# Autodesk Inventor assembly: Full Project Assembly
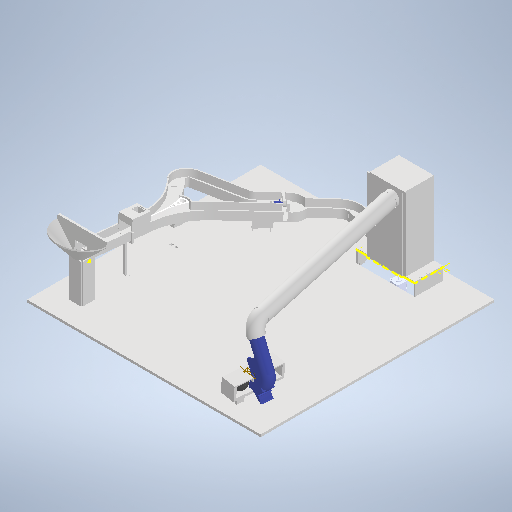
[picture p0: Inventor's stored thumbnail of the model, 512x512]
Saved by Autodesk Inventor 2025.3 (Build 293356000, 356)
## iProperties
Created: 2026-04-18
Part Number: Full Project Assembly
Document SubType Name: Assembly
Designer: kamal
Author: kamal
## Documents named in this file (21)
- C:\Users\kamal\OneDrive\Desktop\Personal\semester 4\Basics of Mechatronics\Full Assembly\Full Project Assembly.iam
- C:\Users\kamal\OneDrive\Desktop\Personal\semester 4\Basics of Mechatronics\Full Assembly\Base.ipt
- C:\Users\kamal\OneDrive\Desktop\Personal\semester 4\Basics of Mechatronics\Full Assembly\Sorting Full Mechanism.iam
- C:\Users\kamal\OneDrive\Desktop\Personal\semester 4\Basics of Mechatronics\Full Assembly\Sorting Holder x1.ipt
- C:\Users\kamal\OneDrive\Desktop\Personal\semester 4\Basics of Mechatronics\Full Assembly\Landing Holder.ipt
- C:\Users\kamal\OneDrive\Desktop\Personal\semester 4\Basics of Mechatronics\Full Assembly\track 1832.ipt
- C:\Users\kamal\OneDrive\Desktop\Personal\semester 4\Basics of Mechatronics\Full Assembly\Collector.ipt
- C:\Users\kamal\OneDrive\Desktop\Personal\semester 4\Basics of Mechatronics\Full Assembly\track z1906.ipt
- C:\Users\kamal\OneDrive\Desktop\Personal\semester 4\Basics of Mechatronics\Full Assembly\selection system 2.iam
- C:\Users\kamal\OneDrive\Desktop\Personal\semester 4\Basics of Mechatronics\Full Assembly\track z2029.ipt
- C:\Users\kamal\OneDrive\Desktop\Personal\semester 4\Basics of Mechatronics\Full Assembly\track z2053.ipt
- C:\Users\kamal\OneDrive\Desktop\Personal\semester 4\Basics of Mechatronics\Full Assembly\track z2059.ipt
- C:\Users\kamal\OneDrive\Desktop\Personal\semester 4\Basics of Mechatronics\Full Assembly\lifting mechanism.iam
- C:\Users\kamal\OneDrive\Desktop\Personal\semester 4\Basics of Mechatronics\Full Assembly\select end track.ipt
- C:\Users\kamal\OneDrive\Desktop\Personal\semester 4\Basics of Mechatronics\Full Assembly\track z2201.ipt
- C:\Users\kamal\OneDrive\Desktop\Personal\semester 4\Basics of Mechatronics\Full Assembly\track z2229.ipt
- C:\Users\kamal\OneDrive\Desktop\Personal\semester 4\Basics of Mechatronics\Full Assembly\SHOOT CAD FINAL.iam
- C:\Users\kamal\OneDrive\Desktop\Personal\semester 4\Basics of Mechatronics\Full Assembly\track z2252.ipt
- C:\Users\kamal\OneDrive\Desktop\Personal\semester 4\Basics of Mechatronics\Full Assembly\track z22522.ipt
- C:\Users\kamal\OneDrive\Desktop\Personal\semester 4\Basics of Mechatronics\Full Assembly\track z2300.ipt
- C:\Users\kamal\OneDrive\Desktop\Personal\semester 4\Basics of Mechatronics\Full Assembly\holder 1.iam
## Components (21 placed, 20 different names)
1. Base:1 — Mate:1, Mate:2, Mate:23, Mate:24, Mate:49, Mate:50, Mate:51
2. Sorting Full Mechanism:1 [sub-assembly] — Mate:4, Mate:5, Mate:6, Mate:12, Mate:13, Mate:14, Mate:21, Mate:22, Mate:25, Mate:26
3. Sorting Holder x1:1 — Mate:1, Mate:2, Mate:4, Mate:5, Mate:6
4. track 1832:1 — Mate:12, Mate:13, Mate:14, Mate:19, Mate:20
5. Collector:1 — Mate:19, Mate:20
6. Landing Holder:1 — Mate:23, Mate:24
7. track z1906:1 — Mate:21, Mate:22, Mate:52, Mate:53
8. selection system 2:1 [sub-assembly] — Mate:27, Mate:28, Mate:41, Mate:42, Mate:54, Mate:55, Mate:56, Mate:57
9. track z2029:1 — Mate:25, Mate:26, Mate:27, Mate:28
10. track z1906:3 — Mate:35, Mate:36, Mate:52, Mate:53
11. track z2053:1 — Mate:35, Mate:36
12. track z2059:1 — Mate:54, Mate:55, Tangent:1
13. lifting mechanism:1 [sub-assembly] — Mate:49, Mate:50, Insert:1
14. select end track:1 — Mate:41, Mate:42, Mate:43, Mate:44
15. track z2201:1 — Mate:43, Mate:44, Mate:47, Mate:48
16. track z2229:1 — Mate:47, Mate:48
17. SHOOT CAD FINAL:1 [sub-assembly] — Mate:51, Insert:4
18. track z2252:1 — Insert:2, Insert:3
19. track z22522:1 — Insert:1, Insert:2
20. track z2300:1 — Insert:3, Insert:4
21. holder 1:1 [sub-assembly] — Mate:56, Mate:57, Tangent:1
## Relationships (40: Mate 35, Insert 4, Tangent 1)
- Mate:1: Base:1 ↔ Sorting Holder x1:1
- Mate:2: Base:1 ↔ Sorting Holder x1:1
- Mate:4: Sorting Full Mechanism:1 ↔ Sorting Holder x1:1
- Mate:5: Sorting Full Mechanism:1 ↔ Sorting Holder x1:1
- Mate:6: Sorting Full Mechanism:1 ↔ Sorting Holder x1:1
- Mate:12: Sorting Full Mechanism:1 ↔ track 1832:1
- Mate:13: Sorting Full Mechanism:1 ↔ track 1832:1
- Mate:14: Sorting Full Mechanism:1 ↔ track 1832:1
- Mate:19: track 1832:1 ↔ Collector:1
- Mate:20: track 1832:1 ↔ Collector:1
- Mate:21: Sorting Full Mechanism:1 ↔ track z1906:1
- Mate:22: Sorting Full Mechanism:1 ↔ track z1906:1
- Mate:23: Base:1 ↔ Landing Holder:1
- Mate:24: Base:1 ↔ Landing Holder:1
- Mate:25: Sorting Full Mechanism:1 ↔ track z2029:1
- Mate:26: Sorting Full Mechanism:1 ↔ track z2029:1
- Mate:27: selection system 2:1 ↔ track z2029:1
- Mate:28: selection system 2:1 ↔ track z2029:1
- Mate:35: track z1906:3 ↔ track z2053:1
- Mate:36: track z1906:3 ↔ track z2053:1
- Mate:41: selection system 2:1 ↔ select end track:1
- Mate:42: selection system 2:1 ↔ select end track:1
- Mate:43: select end track:1 ↔ track z2201:1
- Mate:44: select end track:1 ↔ track z2201:1
- Mate:47: track z2201:1 ↔ track z2229:1
- Mate:48: track z2201:1 ↔ track z2229:1
- Mate:49: Base:1 ↔ lifting mechanism:1
- Mate:50: Base:1 ↔ lifting mechanism:1
- Mate:51: Base:1 ↔ SHOOT CAD FINAL:1
- Insert:1: lifting mechanism:1 ↔ track z22522:1
- Insert:2: track z2252:1 ↔ track z22522:1
- Insert:3: track z2252:1 ↔ track z2300:1
- Insert:4: SHOOT CAD FINAL:1 ↔ track z2300:1
- Mate:52: track z1906:1 ↔ track z1906:3
- Mate:53: track z1906:1 ↔ track z1906:3
- Mate:54: selection system 2:1 ↔ track z2059:1
- Mate:55: selection system 2:1 ↔ track z2059:1
- Mate:56: selection system 2:1 ↔ holder 1:1
- Mate:57: selection system 2:1 ↔ holder 1:1
- Tangent:1: track z2059:1 ↔ holder 1:1
